# Autodesk Inventor assembly: A1-19010-100-00 N6 nozzle insert
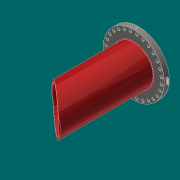
[picture p0: Inventor's stored thumbnail of the model, 180x180]
Saved by Autodesk Inventor 2017.3 (Build 213257000, 257)
## iProperties
Created: 2014-07-18
Part Number: A1-19010-100-00 N6 nozzle insert
Document SubType Name: Weldment
Designer: Graeme_Van_Dongen
Weld Material: Steel, Mild, Welded
Mass: 1.08806e+06 g
Surface Area: 84570.1 cm^2
Volume: 146510 cm^3
Density: 7.42648 g/cm^3
Author: Graeme_Van_Dongen
## Documents named in this file (6)
- N:\A1 - Projects\A1-19\A1-19010--Suncor HCWI N6 N7 nozzle insert\A1-19010-100-00 N6 nozzle insert.iam
- N:\A1 - Projects\A1-19\A1-19010--Suncor HCWI N6 N7 nozzle insert\A1-19010-100-03 Tab - SHORT.ipt
- N:\A1 - Projects\A1-19\A1-19010--Suncor HCWI N6 N7 nozzle insert\A1-19010-100-04 Tab - LONG.ipt
- N:\Inventor\Content Center Files\R2017\en-US\ANSI B18.3(08)\ANSI B18.3 - 3_4-10 UNC - 0.75(24).ipt
- N:\A1 - Projects\A1-19\A1-19010--Suncor HCWI N6 N7 nozzle insert\A1-19010-100-01 30in CL300 RFBL flange.ipt
- N:\A1 - Projects\A1-19\A1-19010--Suncor HCWI N6 N7 nozzle insert\A1-19010-100-02 HCWI nozzle insert.ipt
## Components (6 placed, 5 different names)
1. A1-19010-100-02 HCWI nozzle insert:1 — Insert:1, Angle:1
2. A1-19010-100-01 30in CL300 RFBL flange:1 — Insert:1, Angle:1, Insert:2, Angle:2, Angle:3, Mate:1, Tangent:1, Angle:4, Angle:5
3. A1-19010-100-03 Tab - SHORT:1 — Insert:2, Angle:2, Insert:3
4. A1-19010-100-04 Tab - LONG:1 — Insert:3, Angle:3
5. Hexagon Socket Set Screw - Flat Point - Inch 3/4-10 UNC x 0.75:1 — Mate:1, Tangent:1, Angle:4, Angle:5
6. Hexagon Socket Set Screw - Flat Point - Inch 3/4-10 UNC x 0.75:2
## Component patterns: (2 elements, first: Hexagon Socket Set Screw - Flat Point - Inch 3/4-10 UNC x 0.75:1)
## Relationships (10: Angle 5, Insert 3, Mate 1, Tangent 1)
- Insert:1: A1-19010-100-02 HCWI nozzle insert:1 ↔ A1-19010-100-01 30in CL300 RFBL flange:1
- Angle:1 (0 deg): A1-19010-100-02 HCWI nozzle insert:1 ↔ A1-19010-100-01 30in CL300 RFBL flange:1
- Insert:2 (41.275 mm): A1-19010-100-01 30in CL300 RFBL flange:1 ↔ A1-19010-100-03 Tab - SHORT:1
- Angle:2 (180 deg): A1-19010-100-01 30in CL300 RFBL flange:1 ↔ A1-19010-100-03 Tab - SHORT:1
- Insert:3: A1-19010-100-03 Tab - SHORT:1 ↔ A1-19010-100-04 Tab - LONG:1
- Angle:3 (0 deg): A1-19010-100-01 30in CL300 RFBL flange:1 ↔ A1-19010-100-04 Tab - LONG:1
- Mate:1: A1-19010-100-01 30in CL300 RFBL flange:1 ↔ Hexagon Socket Set Screw - Flat Point - Inch 3/4-10 UNC x 0.75:1
- Tangent:1: A1-19010-100-01 30in CL300 RFBL flange:1 ↔ Hexagon Socket Set Screw - Flat Point - Inch 3/4-10 UNC x 0.75:1
- Angle:4 (0 deg): A1-19010-100-01 30in CL300 RFBL flange:1 ↔ Hexagon Socket Set Screw - Flat Point - Inch 3/4-10 UNC x 0.75:1
- Angle:5 (0 deg): A1-19010-100-01 30in CL300 RFBL flange:1 ↔ Hexagon Socket Set Screw - Flat Point - Inch 3/4-10 UNC x 0.75:1
